# Autodesk Inventor assembly: ASSEMBLY_Nut_Knob
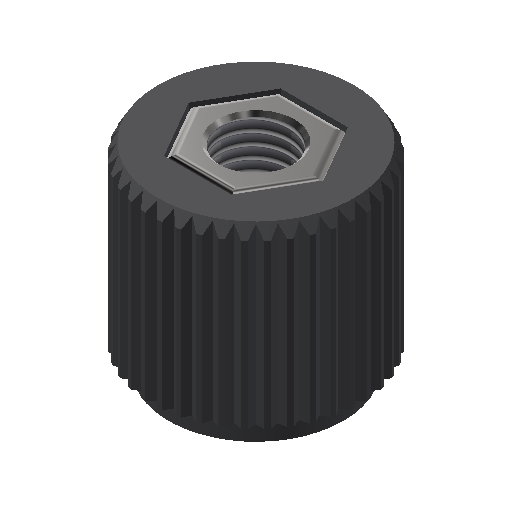
[picture p0: Inventor's stored thumbnail of the model, 512x512]
Saved by Autodesk Inventor 2025 (Build 290162010, 162A)
## iProperties
Created: 2018-02-17
Part Number: ASSEMBLY_Nut_Knob
Material: Ogólny
Document SubType Name: Assembly
Designer: Andrzej
Mass: 3.50402 g
Surface Area: 23.2248 cm^2
Volume: 3.50402 cm^3
Density: 1 g/cm^3
Author: Andrzej
## Documents named in this file (3)
- D:\_ANDRZEJ_LACZEWSKI\_OTHER\MECH - 3D Printed PCB Vise\MCAD\1_REV1\ASSEMBLY_MAIN_REVA\ASSEMBLY_Nut_Knob.iam
- D:\_ANDRZEJ_LACZEWSKI\_OTHER\MECH - 3D Printed PCB Vise\MCAD\1_REV1\__COTS_PARTS\COTS_GENERIC_M6_Nut.ipt
- D:\_ANDRZEJ_LACZEWSKI\_OTHER\MECH - 3D Printed PCB Vise\MCAD\1_REV1\ASSEMBLY_MAIN_REVA\3DP_ABS_Nut_Knob.ipt
## Components (2 placed, 2 different names)
1. COTS_GENERIC_M6_Nut:1 — Zestawiający:1, Zestawiający:2
2. 3DP_ABS_Nut_Knob:1 — Zestawiający:1, Zestawiający:2
## Relationships (2: Mate 2)
- Zestawiający:1 [Mate]: COTS_GENERIC_M6_Nut:1 ↔ 3DP_ABS_Nut_Knob:1
- Zestawiający:2 [Mate]: COTS_GENERIC_M6_Nut:1 ↔ 3DP_ABS_Nut_Knob:1
